# Autodesk Inventor assembly: BV-ASM-222-100
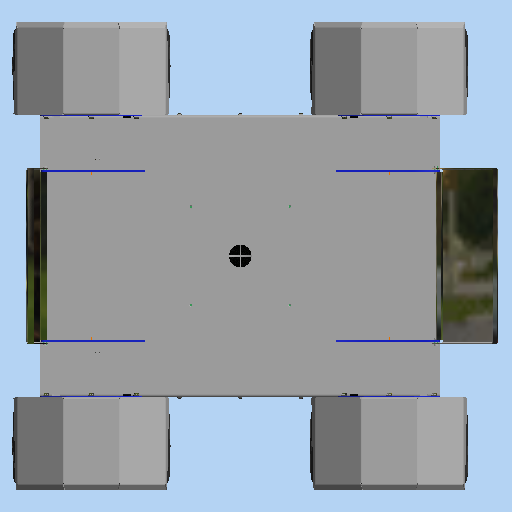
[picture p0: Inventor's stored thumbnail of the model, 512x512]
Saved by Autodesk Inventor 2025.3 (Build 293356030, 356C)
## iProperties
Created: 2025-12-05
Part Number: BV-ASM-222-100
Document SubType Name: Assembly
Designer: josh
Mass: 407870 g
Surface Area: 199043 cm^2
Volume: 211268 cm^3
Density: 1.93058 g/cm^3
Description: BASE VEHICLE COMPLETE ASSEMBLY
Author: josh
## iProperties of the stored document MemberDocs/xFojfi5agHc25u2sk4sonpsnbLc
Created: 2025-12-05
Document SubType Name: Assembly
Designer: josh
Mass: 407870 g
Surface Area: 199043 cm^2
Volume: 211268 cm^3
Density: 1.93058 g/cm^3
Description: BASE VEHICLE COMPLETE ASSEMBLY
Author: josh
## iProperties of the stored document MemberDocs/x54frrunuJ0si20qmEdadrqylTg
Created: 2025-12-05
Document SubType Name: Assembly
Designer: josh
Mass: 407870 g
Surface Area: 199043 cm^2
Volume: 211268 cm^3
Density: 1.93058 g/cm^3
Description: BASE VEHICLE COMPLETE ASSEMBLY
Author: josh
## iProperties of the stored document MemberDocs/xWsksy4mhNck53lhqBkerg4h2Mb
Created: 2025-12-05
Document SubType Name: Assembly
Designer: josh
Mass: 407870 g
Surface Area: 199043 cm^2
Volume: 211268 cm^3
Density: 1.93058 g/cm^3
Description: BASE VEHICLE COMPLETE ASSEMBLY
Author: josh
## Documents named in this file (54)
- R:\A1- Neuweg Design Data\OM Robotics\BASE VEHICLE DESIGN PROJECT\BV-ASM-222-100.iam
- R:\A1- Neuweg Design Data\OM Robotics\BASE VEHICLE DESIGN PROJECT\BV-222-105.ipt
- R:\A1- Neuweg Design Data\OM Robotics\BASE VEHICLE DESIGN PROJECT\BV-222-108.ipt
- R:\A1- Neuweg Design Data\OM Robotics\BASE VEHICLE DESIGN PROJECT\BV-222-112.ipt
- R:\A1- Neuweg Design Data\OM Robotics\BASE VEHICLE DESIGN PROJECT\BV-222-119.ipt
- R:\A1- Neuweg Design Data\OM Robotics\BASE VEHICLE DESIGN PROJECT\BV-222-120.ipt
- R:\A1- Neuweg Design Data\OM Robotics\BASE VEHICLE DESIGN PROJECT\0222-110.ipt
- R:\A1- Neuweg Design Data\OM Robotics\BASE VEHICLE DESIGN PROJECT\3_8-16 x 5_8 Flange Bolt.ipt
- R:\A1- Neuweg Design Data\OM Robotics\BASE VEHICLE DESIGN PROJECT\1_4-20 UNC x 0.625.ipt
- R:\A1- Neuweg Design Data\OM Robotics\BASE VEHICLE DESIGN PROJECT\90128A277.ipt
- R:\A1- Neuweg Design Data\OM Robotics\BASE VEHICLE DESIGN PROJECT\91290A446.ipt
- R:\A1- Neuweg Design Data\OM Robotics\BASE VEHICLE DESIGN PROJECT\91259A177.ipt
- R:\A1- Neuweg Design Data\OM Robotics\BASE VEHICLE DESIGN PROJECT\94945A213.ipt
- R:\A1- Neuweg Design Data\OM Robotics\BASE VEHICLE DESIGN PROJECT\BV-ASM-222-102.iam
- R:\A1- Neuweg Design Data\OM Robotics\BASE VEHICLE DESIGN PROJECT\30205.ipt
- R:\A1- Neuweg Design Data\OM Robotics\BASE VEHICLE DESIGN PROJECT\251105 Motor_Drive.ipt
- R:\A1- Neuweg Design Data\OM Robotics\BASE VEHICLE DESIGN PROJECT\22x10x8.ipt
- R:\A1- Neuweg Design Data\OM Robotics\BASE VEHICLE DESIGN PROJECT\0222-113-2.ipt
- R:\A1- Neuweg Design Data\OM Robotics\BASE VEHICLE DESIGN PROJECT\97260A109.ipt
- R:\A1- Neuweg Design Data\OM Robotics\BASE VEHICLE DESIGN PROJECT\1199N323.ipt
- R:\A1- Neuweg Design Data\OM Robotics\BASE VEHICLE DESIGN PROJECT\BV-ASM-222-103.iam
- R:\A1- Neuweg Design Data\OM Robotics\BASE VEHICLE DESIGN PROJECT\BV-ASM-222-106.iam
- R:\A1- Neuweg Design Data\OM Robotics\BASE VEHICLE DESIGN PROJECT\0222-113.ipt
- R:\A1- Neuweg Design Data\OM Robotics\BASE VEHICLE DESIGN PROJECT\96717A416.ipt
- R:\A1- Neuweg Design Data\OM Robotics\BASE VEHICLE DESIGN PROJECT\4991T961.ipt
- C:\WORK\INVENTOR PROJECTS\misc custom projects\O&M ROBOTICS\ROBOT BASE VEHICLE\BV-222-105.ipt
- C:\WORK\INVENTOR PROJECTS\misc custom projects\O&M ROBOTICS\ROBOT BASE VEHICLE\BV-222-106.ipt
- C:\WORK\INVENTOR PROJECTS\misc custom projects\O&M ROBOTICS\ROBOT BASE VEHICLE\BV-222-107.ipt
- C:\WORK\INVENTOR PROJECTS\misc custom projects\O&M ROBOTICS\ROBOT BASE VEHICLE\BV-222-108.ipt
- C:\WORK\INVENTOR PROJECTS\misc custom projects\O&M ROBOTICS\ROBOT BASE VEHICLE\BV-222-109.ipt
- C:\WORK\INVENTOR PROJECTS\misc custom projects\O&M ROBOTICS\ROBOT BASE VEHICLE\BV-222-112.ipt
- C:\WORK\INVENTOR PROJECTS\misc custom projects\O&M ROBOTICS\ROBOT BASE VEHICLE\BV-222-116.ipt
- C:\WORK\INVENTOR PROJECTS\misc custom projects\O&M ROBOTICS\ROBOT BASE VEHICLE\BV-222-117.ipt
- C:\WORK\INVENTOR PROJECTS\misc custom projects\O&M ROBOTICS\ROBOT BASE VEHICLE\BV-222-118.ipt
- C:\WORK\INVENTOR PROJECTS\misc custom projects\O&M ROBOTICS\ROBOT BASE VEHICLE\BV-222-119.ipt
- C:\WORK\INVENTOR PROJECTS\misc custom projects\O&M ROBOTICS\ROBOT BASE VEHICLE\BV-222-120.ipt
- C:\WORK\INVENTOR PROJECTS\misc custom projects\O&M ROBOTICS\ROBOT BASE VEHICLE\0222-110.ipt
- C:\WORK\INVENTOR PROJECTS\misc custom projects\O&M ROBOTICS\ROBOT BASE VEHICLE\3_8-16 x 5_8 Flange Bolt.ipt
- C:\WORK\INVENTOR PROJECTS\misc custom projects\O&M ROBOTICS\ROBOT BASE VEHICLE\1_4-20 UNC x 0.625.ipt
- C:\WORK\INVENTOR PROJECTS\misc custom projects\O&M ROBOTICS\ROBOT BASE VEHICLE\90128A277\90128A277\90128A277.ipt
- C:\WORK\INVENTOR PROJECTS\misc custom projects\O&M ROBOTICS\ROBOT BASE VEHICLE\91290A446\91290A446\91290A446.ipt
- C:\WORK\INVENTOR PROJECTS\misc custom projects\O&M ROBOTICS\ROBOT BASE VEHICLE\91259A177\91259A177\91259A177.ipt
- C:\WORK\INVENTOR PROJECTS\misc custom projects\O&M ROBOTICS\ROBOT BASE VEHICLE\94945A213\94945A213\94945A213.ipt
- C:\WORK\INVENTOR PROJECTS\misc custom projects\O&M ROBOTICS\ROBOT BASE VEHICLE\BV-ASM-222-102.iam
- C:\WORK\INVENTOR PROJECTS\misc custom projects\O&M ROBOTICS\ROBOT BASE VEHICLE\30205\30205\30205.ipt
- C:\WORK\INVENTOR PROJECTS\misc custom projects\O&M ROBOTICS\ROBOT BASE VEHICLE\251105 Motor_Drive.ipt
- C:\WORK\INVENTOR PROJECTS\misc custom projects\O&M ROBOTICS\ROBOT BASE VEHICLE\22x10x8.ipt
- C:\WORK\INVENTOR PROJECTS\misc custom projects\O&M ROBOTICS\ROBOT BASE VEHICLE\0222-113-2.ipt
- C:\WORK\INVENTOR PROJECTS\misc custom projects\O&M ROBOTICS\ROBOT BASE VEHICLE\97260A109.ipt
- C:\WORK\INVENTOR PROJECTS\misc custom projects\O&M ROBOTICS\ROBOT BASE VEHICLE\93560A112_Steel Hex Weld Nut\93560A112_Steel Hex Weld Nut\93560A112.ipt
- C:\WORK\INVENTOR PROJECTS\misc custom projects\O&M ROBOTICS\ROBOT BASE VEHICLE\1199N323\1199N323\1199N323.ipt
- C:\WORK\INVENTOR PROJECTS\misc custom projects\O&M ROBOTICS\ROBOT BASE VEHICLE\BV-ASM-222-103.iam
- C:\WORK\INVENTOR PROJECTS\misc custom projects\O&M ROBOTICS\ROBOT BASE VEHICLE\BV-ASM-222-104.iam
- C:\WORK\INVENTOR PROJECTS\misc custom projects\O&M ROBOTICS\ROBOT BASE VEHICLE\BV-ASM-222-105.iam
## Components (194 placed, 24 different names)
1. BV-ASM-222-106:1 [sub-assembly] — Insert:95, Insert:96, Insert:97, Insert:98, Insert:99, Insert:100, Insert:101, Insert:102, Insert:103, Insert:104, Insert:129, Insert:130, Insert:131, Insert:132, Insert:133, Insert:134, Insert:135, Insert:136, Insert:137, Insert:138, Insert:139, Insert:140, Insert:141, Insert:142, Insert:143, Insert:144, Mate:105, Mate:107, Mate:108, Mate:109, Mate:111, Mate:113, Mate:114, Mate:116, Mate:118, Mate:120, Mate:122, Mate:123, Mate:124, Insert:221, Insert:222, Insert:223, Mate:125, Mate:126, Mate:127, Insert:226, Insert:227, Insert:228, Mate:128, Mate:129, Mate:130, Insert:231, Insert:232, Insert:233, Mate:131, Mate:132, Mate:133, Insert:234, Insert:235, Insert:236, Flush:20, Mate:134, Insert:238, Insert:240, Mate:136, Insert:243, Insert:244, Insert:245, Insert:246, Insert:247, Insert:248, Insert:249, Insert:250, Insert:252, Insert:253, Insert:254, Insert:255, Insert:256, Insert:257, Insert:258, Insert:259, Insert:260, Insert:261, Insert:262, Insert:263, Insert:264, Insert:265, Insert:266, Insert:267, Insert:268, Insert:269, Insert:270, Insert:271, Insert:272, Insert:273
2. BV-ASM-222-103:1 [sub-assembly] — Flush:8, Flush:9, Flush:10, Mate:131, Mate:132, Mate:133
3. BV-ASM-222-103:2 [sub-assembly] — Insert:205, Insert:206, Mate:128, Mate:129, Mate:130, Insert:229, Insert:230
4. BV-ASM-222-103:3 [sub-assembly] — Insert:209, Insert:210, Mate:125, Mate:126, Mate:127, Insert:224, Insert:225
5. BV-ASM-222-103:4 [sub-assembly] — Insert:213, Insert:214, Mate:122, Mate:123, Mate:124, Insert:219, Insert:220
6. BV-222-105:1 — Insert:117, Insert:118, Insert:119, Insert:120, Insert:121, Insert:122, Insert:123, Insert:124, Insert:125, Insert:126, Insert:127, Insert:128
7. BV-222-108:1 — Flush:1, Mate:3, Mate:135, Mate:136
8. BV-222-112:1 — Mate:73, Mate:74, Mate:75, Mate:76, Mate:77, Mate:78, Mate:79, Mate:80, Mate:81, Mate:82, Mate:83, Mate:84, Mate:85, Mate:86, Mate:87, Mate:88, Mate:89, Mate:90, Mate:91, Mate:92
9. BV-222-119:1 — Insert:175, Insert:190
10. BV-222-120:1 — Mate:5
11. BV-222-112:3
12. BV-222-108:2 — Mate:3, Flush:20, Mate:134, Mate:135
13. BV-222-119:2 — Insert:176, Insert:186
14. BV-222-120:2
15. BV-222-119:3 — Insert:169, Insert:191
16. BV-222-120:3 — Mate:14
17. BV-222-119:4 — Insert:171, Insert:187
18. BV-222-120:4 — Mate:11
19. BV-ASM-222-102:1 [sub-assembly] — Mate:12, Mate:13, Insert:30, Insert:31, Insert:215, Insert:275, Mate:141, Flush:25, Mate:142
20. BV-ASM-222-102:2 [sub-assembly] — Mate:4, Mate:6, Insert:16, Insert:17, Mate:102, Insert:217, Insert:276, Mate:139, Flush:21, Flush:22
21. BV-ASM-222-102:3 [sub-assembly] — Mate:9, Mate:10, Insert:28, Insert:29, Mate:103, Mate:137, Mate:138, Insert:274, Mate:143, Flush:26, Flush:27
22. BV-ASM-222-102:4 [sub-assembly] — Mate:7, Mate:8, Insert:22, Insert:23, Mate:101, Insert:216, Insert:277, Mate:140, Flush:23, Flush:24
23. 251105 Motor_Drive:1 — Mate:4, Mate:5, Mate:6, Flush:2, Flush:3, Mate:102
24. 22x10x8:1 — Insert:16, Insert:17, Insert:280
25. 97260A109:1 — Insert:196
26. 251105 Motor_Drive:2 — Mate:7, Flush:2, Flush:3, Mate:8, Flush:4, Mate:101
27. 97260A109:2 — Insert:194
28. 22x10x8:2 — Insert:22, Insert:23, Insert:281
29. 251105 Motor_Drive:3 — Mate:9, Mate:10, Mate:11, Flush:4, Flush:5, Mate:103
30. 251105 Motor_Drive:4 — Mate:12, Mate:13, Mate:14, Flush:5
31. 97260A109:3 — Insert:200
32. 97260A109:4 — Insert:198
33. 22x10x8:3 — Insert:28, Insert:29, Insert:278
34. 22x10x8:4 — Insert:30, Insert:31, Insert:279
35. 0222-110:1 — Mate:104, Flush:7, Mate:106, Mate:107, Mate:108, Mate:110, Mate:112
36. 0222-110:2 — Flush:7, Flush:19, Mate:113, Mate:115, Mate:117, Mate:119, Mate:121
37. Hex Flange Screw - Inch (IFI) 3/8-16 UNC x 0.625:9 — Mate:120, Mate:121
38. Hex Flange Screw - Inch (IFI) 3/8-16 UNC x 0.625:10 — Mate:118, Mate:119
39. Hex Flange Screw - Inch (IFI) 3/8-16 UNC x 0.625:11 — Mate:116, Mate:117
40. Hex Flange Screw - Inch (IFI) 3/8-16 UNC x 0.625:12 — Mate:114, Mate:115
41. Hex Flange Screw - Inch (IFI) 3/8-16 UNC x 0.625:13 — Mate:105, Mate:106
42. Hex Flange Screw - Inch (IFI) 3/8-16 UNC x 0.625:14 — Mate:109, Mate:110
43. Hex Flange Screw - Inch (IFI) 3/8-16 UNC x 0.625:15
44. Hex Flange Screw - Inch (IFI) 3/8-16 UNC x 0.625:16 — Mate:111, Mate:112
45. Hex Flange Screw - Inch (IFI) 3/8-16 UNC x 0.625:18 — Mate:21, Mate:22, Insert:236
46. Hex Flange Screw - Inch (IFI) 3/8-16 UNC x 0.625:19 — Mate:21, Mate:22, Insert:235
47. Hex Flange Screw - Inch (IFI) 3/8-16 UNC x 0.625:20 — Mate:23, Mate:24, Insert:234
48. Hex Flange Screw - Inch (IFI) 3/8-16 UNC x 0.625:21 — Mate:23, Mate:24, Insert:231
49. Hex Flange Screw - Inch (IFI) 3/8-16 UNC x 0.625:22 — Mate:25, Mate:26, Insert:232
50. Hex Flange Screw - Inch (IFI) 3/8-16 UNC x 0.625:23 — Mate:25, Mate:26, Insert:233
51. Hex Flange Screw - Inch (IFI) 3/8-16 UNC x 0.625:24 — Mate:27, Mate:28, Insert:221
52. Hex Flange Screw - Inch (IFI) 3/8-16 UNC x 0.625:25 — Mate:27, Mate:28, Insert:223
53. Hex Flange Screw - Inch (IFI) 3/8-16 UNC x 0.625:26 — Mate:29, Mate:30, Insert:222
54. Hex Flange Screw - Inch (IFI) 3/8-16 UNC x 0.625:27 — Mate:29, Mate:30, Insert:226
55. Hex Flange Screw - Inch (IFI) 3/8-16 UNC x 0.625:28 — Mate:31, Mate:32, Insert:227
56. Hex Flange Screw - Inch (IFI) 3/8-16 UNC x 0.625:29 — Mate:31, Mate:32, Insert:228
57. Hex Flange Screw - Inch (IFI) 3/8-16 UNC x 0.625:30 — Mate:33, Mate:34
58. Hex Flange Screw - Inch (IFI) 3/8-16 UNC x 0.625:31 — Mate:33, Mate:34
59. Hex Flange Screw - Inch (IFI) 3/8-16 UNC x 0.625:32 — Mate:35, Mate:36, Insert:205, Insert:230
60. Hex Flange Screw - Inch (IFI) 3/8-16 UNC x 0.625:33 — Mate:35, Mate:36, Insert:206, Insert:229
61. Hex Flange Screw - Inch (IFI) 3/8-16 UNC x 0.625:34 — Mate:37, Mate:38, Insert:214, Insert:220
62. Hex Flange Screw - Inch (IFI) 3/8-16 UNC x 0.625:35 — Mate:37, Mate:38, Insert:213, Insert:219
63. Hex Flange Screw - Inch (IFI) 3/8-16 UNC x 0.625:36 — Mate:39, Mate:40, Insert:209, Insert:224
64. Hex Flange Screw - Inch (IFI) 3/8-16 UNC x 0.625:37 — Mate:39, Mate:40, Insert:210, Insert:225
65. 1_4-20 UNC x 0.625:1 — Insert:95, Mate:41, Mate:42
66. 1_4-20 UNC x 0.625:2 — Insert:96, Mate:41, Mate:42
67. 1_4-20 UNC x 0.625:3 — Insert:97, Mate:43, Mate:44
68. 1_4-20 UNC x 0.625:4 — Insert:98, Mate:43, Mate:44
69. 1_4-20 UNC x 0.625:5 — Insert:99, Mate:45, Mate:46
70. 1_4-20 UNC x 0.625:6 — Insert:100, Mate:45, Mate:46
71. 1_4-20 UNC x 0.625:7 — Insert:101, Mate:47, Mate:48
72. 1_4-20 UNC x 0.625:8 — Insert:102, Mate:47, Mate:48
73. 1_4-20 UNC x 0.625:9 — Insert:103, Mate:49, Mate:50
74. 1_4-20 UNC x 0.625:10 — Insert:104, Mate:49, Mate:50
75. Hex Flange Screw - Inch (IFI) 3/8-16 UNC x 0.625:38 — Insert:117, Mate:51, Mate:52
76. Hex Flange Screw - Inch (IFI) 3/8-16 UNC x 0.625:39 — Insert:118, Mate:51, Mate:52
77. Hex Flange Screw - Inch (IFI) 3/8-16 UNC x 0.625:40 — Insert:119, Mate:53, Mate:54
78. Hex Flange Screw - Inch (IFI) 3/8-16 UNC x 0.625:41 — Insert:120, Mate:53, Mate:54
79. Hex Flange Screw - Inch (IFI) 3/8-16 UNC x 0.625:42 — Insert:121, Mate:55, Mate:56
80. Hex Flange Screw - Inch (IFI) 3/8-16 UNC x 0.625:43 — Insert:122, Mate:55, Mate:56
81. Hex Flange Screw - Inch (IFI) 3/8-16 UNC x 0.625:44 — Insert:123, Mate:57, Mate:58
82. Hex Flange Screw - Inch (IFI) 3/8-16 UNC x 0.625:45 — Insert:124, Mate:57, Mate:58
83. Hex Flange Screw - Inch (IFI) 3/8-16 UNC x 0.625:46 — Insert:125, Mate:59, Mate:60
84. Hex Flange Screw - Inch (IFI) 3/8-16 UNC x 0.625:47 — Insert:126, Mate:59, Mate:60
85. Hex Flange Screw - Inch (IFI) 3/8-16 UNC x 0.625:48 — Insert:127, Mate:61, Mate:62
86. Hex Flange Screw - Inch (IFI) 3/8-16 UNC x 0.625:49 — Insert:128, Mate:61, Mate:62
87. 1_4-20 UNC x 0.625:11 — Mate:75, Mate:76
88. 1_4-20 UNC x 0.625:12 — Mate:89, Mate:90
89. 1_4-20 UNC x 0.625:13 — Mate:77, Mate:78
90. 1_4-20 UNC x 0.625:14 — Mate:81, Mate:82
91. 1_4-20 UNC x 0.625:15 — Mate:79, Mate:80
92. 1_4-20 UNC x 0.625:16 — Mate:91, Mate:92
93. 1_4-20 UNC x 0.625:17 — Mate:85, Mate:86
94. 1_4-20 UNC x 0.625:18 — Mate:83, Mate:84
95. 1_4-20 UNC x 0.625:19 — Mate:87, Mate:88
96. 1_4-20 UNC x 0.625:20 — Mate:73, Mate:74
97. 1_4-20 UNC x 0.625:21 — Mate:93, Mate:94
98. 1_4-20 UNC x 0.625:22 — Mate:93, Mate:94
99. 1_4-20 UNC x 0.625:23 — Mate:95, Mate:96
100. 1_4-20 UNC x 0.625:24 — Mate:95, Mate:96
101. 1_4-20 UNC x 0.625:25
102. 1_4-20 UNC x 0.625:26
103. 1_4-20 UNC x 0.625:27 — Mate:97, Mate:98
104. 1_4-20 UNC x 0.625:28 — Mate:97, Mate:98
105. 1_4-20 UNC x 0.625:29 — Mate:99, Mate:100
106. 1_4-20 UNC x 0.625:30 — Mate:99, Mate:100
107. 90128A277:1 — Insert:129
108. 90128A277:2 — Insert:130
109. 90128A277:3 — Insert:131
110. 90128A277:4 — Insert:132
111. 90128A277:5 — Insert:133
112. 90128A277:6 — Insert:134
113. 90128A277:7 — Insert:135
114. 90128A277:8 — Insert:136
115. 90128A277:9 — Insert:137
116. 90128A277:10 — Insert:138
117. 90128A277:11 — Insert:139
118. 90128A277:12 — Insert:140
119. 90128A277:13 — Insert:141
120. 90128A277:14 — Insert:142
121. 90128A277:15 — Insert:143
122. 90128A277:16 — Insert:144
123. 91290A446:1 — Insert:273
124. 91290A446:2 — Insert:271
125. 91290A446:3 — Insert:272
126. 91290A446:4 — Insert:270
127. 91290A446:5 — Insert:260
128. 91290A446:6 — Insert:259
129. 91290A446:7 — Insert:261
130. 91290A446:8 — Insert:258
131. 91290A446:9 — Insert:265
132. 91290A446:10 — Insert:264
133. 91290A446:11 — Insert:262
134. 91290A446:12 — Insert:263
135. 91290A446:13 — Insert:269
136. 91290A446:14 — Insert:268
137. 91290A446:15 — Insert:267
138. 91290A446:16 — Insert:266
139. 91259A177:1 — Insert:244
140. 91259A177:2 — Insert:245
141. 91259A177:3 — Insert:247
142. 91259A177:4 — Insert:248
143. 94945A213:1 — Insert:246
144. 94945A213:2 — Insert:243
145. 94945A213:3 — Insert:238
146. 94945A213:4 — Insert:240
147. 30205:1 — Insert:215, Insert:249
148. 30205:2 — Insert:169, Insert:197
149. 30205:3 — Insert:255, Mate:137, Mate:138
150. 30205:4 — Insert:171, Insert:199
151. 30205:5 — Insert:176, Insert:193
152. 30205:6 — Insert:216, Insert:253
153. 30205:7 — Insert:175, Insert:195
154. 30205:8 — Insert:217, Insert:256
155. 0222-113-2:1 — Insert:199, Insert:200
156. 0222-113-2:2 — Insert:193, Insert:194
157. 0222-113-2:3 — Insert:197, Insert:198
158. 0222-113-2:4 — Insert:195, Insert:196
159. 1199N323:1 — Insert:254
160. 1199N323:2 — Insert:186
161. 1199N323:3 — Insert:187
162. 1199N323:4 — Insert:252
163. 1199N323:5 — Insert:257
164. 1199N323:6 — Insert:190
165. 1199N323:7 — Insert:191
166. 1199N323:8 — Insert:250
167. 0222-113:1 — Insert:274
168. 0222-113:2 — Insert:275
169. 0222-113:3 — Insert:276
170. 0222-113:4 — Insert:277
171. 96717A416:1 — Mate:139, Flush:21, Flush:22
172. 96717A416:2 — Mate:140, Flush:23, Flush:24
173. 96717A416:3 — Mate:141, Flush:25, Mate:142
174. 96717A416:4 — Mate:143, Flush:26, Flush:27
175. 4991T961:1 — Insert:278
176. 4991T961:2
177. 4991T961:3
178. 4991T961:4
179. 4991T961:5
180. 4991T961:6 — Insert:279
181. 4991T961:7
182. 4991T961:8
183. 4991T961:9
184. 4991T961:10
185. 4991T961:11 — Insert:280
186. 4991T961:12
187. 4991T961:13
188. 4991T961:14
189. 4991T961:15
190. 4991T961:16 — Insert:281
191. 4991T961:17
192. 4991T961:18
193. 4991T961:19
194. 4991T961:20
## Component patterns: (5 elements, first: 4991T961:1), (5 elements, first: 4991T961:6), (5 elements, first: 4991T961:11), (5 elements, first: 4991T961:16)
## Relationships (287: Insert 133, Mate 133, Flush 21)
- [Insert]: BV-ASM-222-106:1 ↔ BV-222-112:3
- [Insert]: BV-ASM-222-106:1 ↔ BV-222-112:3
- Flush:1: BV-222-108:1
- Mate:3: BV-222-108:1 ↔ BV-222-108:2
- Mate:4: BV-ASM-222-102:2 ↔ 251105 Motor_Drive:1
- Mate:5: BV-222-120:1 ↔ 251105 Motor_Drive:1
- Mate:6: BV-ASM-222-102:2 ↔ 251105 Motor_Drive:1
- Insert:16: BV-ASM-222-102:2 ↔ 22x10x8:1
- Insert:17: BV-ASM-222-102:2 ↔ 22x10x8:1
- Mate:7: BV-ASM-222-102:4 ↔ 251105 Motor_Drive:2
- Flush:2: 251105 Motor_Drive:1 ↔ 251105 Motor_Drive:2
- Flush:3: 251105 Motor_Drive:1 ↔ 251105 Motor_Drive:2
- Mate:8: BV-ASM-222-102:4 ↔ 251105 Motor_Drive:2
- Insert:22: BV-ASM-222-102:4 ↔ 22x10x8:2
- Insert:23: BV-ASM-222-102:4 ↔ 22x10x8:2
- Mate:9: BV-ASM-222-102:3 ↔ 251105 Motor_Drive:3
- Mate:10: BV-ASM-222-102:3 ↔ 251105 Motor_Drive:3
- Mate:11: BV-222-120:4 ↔ 251105 Motor_Drive:3
- Flush:4: 251105 Motor_Drive:2 ↔ 251105 Motor_Drive:3
- Mate:12: BV-ASM-222-102:1 ↔ 251105 Motor_Drive:4
- Mate:13: BV-ASM-222-102:1 ↔ 251105 Motor_Drive:4
- Mate:14: BV-222-120:3 ↔ 251105 Motor_Drive:4
- Flush:5: 251105 Motor_Drive:3 ↔ 251105 Motor_Drive:4
- Insert:28: BV-ASM-222-102:3 ↔ 22x10x8:3
- Insert:29: BV-ASM-222-102:3 ↔ 22x10x8:3
- Insert:30: BV-ASM-222-102:1 ↔ 22x10x8:4
- Insert:31: BV-ASM-222-102:1 ↔ 22x10x8:4
- Mate:104: 0222-110:1
- Flush:7: 0222-110:1 ↔ 0222-110:2
- Flush:19: 0222-110:2
- Mate:21: Hex Flange Screw - Inch (IFI) 3/8-16 UNC x 0.625:18 ↔ Hex Flange Screw - Inch (IFI) 3/8-16 UNC x 0.625:19
- Mate:22: Hex Flange Screw - Inch (IFI) 3/8-16 UNC x 0.625:18 ↔ Hex Flange Screw - Inch (IFI) 3/8-16 UNC x 0.625:19
- Mate:23: Hex Flange Screw - Inch (IFI) 3/8-16 UNC x 0.625:20 ↔ Hex Flange Screw - Inch (IFI) 3/8-16 UNC x 0.625:21
- Mate:24: Hex Flange Screw - Inch (IFI) 3/8-16 UNC x 0.625:20 ↔ Hex Flange Screw - Inch (IFI) 3/8-16 UNC x 0.625:21
- Mate:25: Hex Flange Screw - Inch (IFI) 3/8-16 UNC x 0.625:22 ↔ Hex Flange Screw - Inch (IFI) 3/8-16 UNC x 0.625:23
- Mate:26: Hex Flange Screw - Inch (IFI) 3/8-16 UNC x 0.625:22 ↔ Hex Flange Screw - Inch (IFI) 3/8-16 UNC x 0.625:23
- Mate:27: Hex Flange Screw - Inch (IFI) 3/8-16 UNC x 0.625:24 ↔ Hex Flange Screw - Inch (IFI) 3/8-16 UNC x 0.625:25
- Mate:28: Hex Flange Screw - Inch (IFI) 3/8-16 UNC x 0.625:24 ↔ Hex Flange Screw - Inch (IFI) 3/8-16 UNC x 0.625:25
- Mate:29: Hex Flange Screw - Inch (IFI) 3/8-16 UNC x 0.625:26 ↔ Hex Flange Screw - Inch (IFI) 3/8-16 UNC x 0.625:27
- Mate:30: Hex Flange Screw - Inch (IFI) 3/8-16 UNC x 0.625:26 ↔ Hex Flange Screw - Inch (IFI) 3/8-16 UNC x 0.625:27
- Mate:31: Hex Flange Screw - Inch (IFI) 3/8-16 UNC x 0.625:28 ↔ Hex Flange Screw - Inch (IFI) 3/8-16 UNC x 0.625:29
- Mate:32: Hex Flange Screw - Inch (IFI) 3/8-16 UNC x 0.625:28 ↔ Hex Flange Screw - Inch (IFI) 3/8-16 UNC x 0.625:29
- [Insert]: BV-ASM-222-103:1 ↔ Hex Flange Screw - Inch (IFI) 3/8-16 UNC x 0.625:30
- [Insert]: BV-ASM-222-103:1 ↔ Hex Flange Screw - Inch (IFI) 3/8-16 UNC x 0.625:31
- Mate:33: Hex Flange Screw - Inch (IFI) 3/8-16 UNC x 0.625:30 ↔ Hex Flange Screw - Inch (IFI) 3/8-16 UNC x 0.625:31
- Mate:34: Hex Flange Screw - Inch (IFI) 3/8-16 UNC x 0.625:30 ↔ Hex Flange Screw - Inch (IFI) 3/8-16 UNC x 0.625:31
- Mate:35: Hex Flange Screw - Inch (IFI) 3/8-16 UNC x 0.625:32 ↔ Hex Flange Screw - Inch (IFI) 3/8-16 UNC x 0.625:33
- Mate:36: Hex Flange Screw - Inch (IFI) 3/8-16 UNC x 0.625:32 ↔ Hex Flange Screw - Inch (IFI) 3/8-16 UNC x 0.625:33
- Mate:37: Hex Flange Screw - Inch (IFI) 3/8-16 UNC x 0.625:34 ↔ Hex Flange Screw - Inch (IFI) 3/8-16 UNC x 0.625:35
- Mate:38: Hex Flange Screw - Inch (IFI) 3/8-16 UNC x 0.625:34 ↔ Hex Flange Screw - Inch (IFI) 3/8-16 UNC x 0.625:35
- Mate:39: Hex Flange Screw - Inch (IFI) 3/8-16 UNC x 0.625:36 ↔ Hex Flange Screw - Inch (IFI) 3/8-16 UNC x 0.625:37
- Mate:40: Hex Flange Screw - Inch (IFI) 3/8-16 UNC x 0.625:36 ↔ Hex Flange Screw - Inch (IFI) 3/8-16 UNC x 0.625:37
- Insert:95: BV-ASM-222-106:1 ↔ 1_4-20 UNC x 0.625:1
- Insert:96: BV-ASM-222-106:1 ↔ 1_4-20 UNC x 0.625:2
- Mate:41: 1_4-20 UNC x 0.625:1 ↔ 1_4-20 UNC x 0.625:2
- Mate:42: 1_4-20 UNC x 0.625:1 ↔ 1_4-20 UNC x 0.625:2
- Insert:97: BV-ASM-222-106:1 ↔ 1_4-20 UNC x 0.625:3
- Insert:98: BV-ASM-222-106:1 ↔ 1_4-20 UNC x 0.625:4
- Mate:43: 1_4-20 UNC x 0.625:3 ↔ 1_4-20 UNC x 0.625:4
- Mate:44: 1_4-20 UNC x 0.625:3 ↔ 1_4-20 UNC x 0.625:4
- Insert:99: BV-ASM-222-106:1 ↔ 1_4-20 UNC x 0.625:5
- Insert:100: BV-ASM-222-106:1 ↔ 1_4-20 UNC x 0.625:6
- Mate:45: 1_4-20 UNC x 0.625:5 ↔ 1_4-20 UNC x 0.625:6
- Mate:46: 1_4-20 UNC x 0.625:5 ↔ 1_4-20 UNC x 0.625:6
- Insert:101: BV-ASM-222-106:1 ↔ 1_4-20 UNC x 0.625:7
- Insert:102: BV-ASM-222-106:1 ↔ 1_4-20 UNC x 0.625:8
- Mate:47: 1_4-20 UNC x 0.625:7 ↔ 1_4-20 UNC x 0.625:8
- Mate:48: 1_4-20 UNC x 0.625:7 ↔ 1_4-20 UNC x 0.625:8
- Insert:103: BV-ASM-222-106:1 ↔ 1_4-20 UNC x 0.625:9
- Insert:104: BV-ASM-222-106:1 ↔ 1_4-20 UNC x 0.625:10
- Mate:49: 1_4-20 UNC x 0.625:9 ↔ 1_4-20 UNC x 0.625:10
- Mate:50: 1_4-20 UNC x 0.625:9 ↔ 1_4-20 UNC x 0.625:10
- Insert:117: BV-222-105:1 ↔ Hex Flange Screw - Inch (IFI) 3/8-16 UNC x 0.625:38
- Insert:118: BV-222-105:1 ↔ Hex Flange Screw - Inch (IFI) 3/8-16 UNC x 0.625:39
- Mate:51: Hex Flange Screw - Inch (IFI) 3/8-16 UNC x 0.625:38 ↔ Hex Flange Screw - Inch (IFI) 3/8-16 UNC x 0.625:39
- Mate:52: Hex Flange Screw - Inch (IFI) 3/8-16 UNC x 0.625:38 ↔ Hex Flange Screw - Inch (IFI) 3/8-16 UNC x 0.625:39
- Insert:119: BV-222-105:1 ↔ Hex Flange Screw - Inch (IFI) 3/8-16 UNC x 0.625:40
- Insert:120: BV-222-105:1 ↔ Hex Flange Screw - Inch (IFI) 3/8-16 UNC x 0.625:41
- Mate:53: Hex Flange Screw - Inch (IFI) 3/8-16 UNC x 0.625:40 ↔ Hex Flange Screw - Inch (IFI) 3/8-16 UNC x 0.625:41
- Mate:54: Hex Flange Screw - Inch (IFI) 3/8-16 UNC x 0.625:40 ↔ Hex Flange Screw - Inch (IFI) 3/8-16 UNC x 0.625:41
- Insert:121: BV-222-105:1 ↔ Hex Flange Screw - Inch (IFI) 3/8-16 UNC x 0.625:42
- Insert:122: BV-222-105:1 ↔ Hex Flange Screw - Inch (IFI) 3/8-16 UNC x 0.625:43
- Mate:55: Hex Flange Screw - Inch (IFI) 3/8-16 UNC x 0.625:42 ↔ Hex Flange Screw - Inch (IFI) 3/8-16 UNC x 0.625:43
- Mate:56: Hex Flange Screw - Inch (IFI) 3/8-16 UNC x 0.625:42 ↔ Hex Flange Screw - Inch (IFI) 3/8-16 UNC x 0.625:43
- Insert:123: BV-222-105:1 ↔ Hex Flange Screw - Inch (IFI) 3/8-16 UNC x 0.625:44
- Insert:124: BV-222-105:1 ↔ Hex Flange Screw - Inch (IFI) 3/8-16 UNC x 0.625:45
- Mate:57: Hex Flange Screw - Inch (IFI) 3/8-16 UNC x 0.625:44 ↔ Hex Flange Screw - Inch (IFI) 3/8-16 UNC x 0.625:45
- Mate:58: Hex Flange Screw - Inch (IFI) 3/8-16 UNC x 0.625:44 ↔ Hex Flange Screw - Inch (IFI) 3/8-16 UNC x 0.625:45
- Insert:125: BV-222-105:1 ↔ Hex Flange Screw - Inch (IFI) 3/8-16 UNC x 0.625:46
- Insert:126: BV-222-105:1 ↔ Hex Flange Screw - Inch (IFI) 3/8-16 UNC x 0.625:47
- Mate:59: Hex Flange Screw - Inch (IFI) 3/8-16 UNC x 0.625:46 ↔ Hex Flange Screw - Inch (IFI) 3/8-16 UNC x 0.625:47
- Mate:60: Hex Flange Screw - Inch (IFI) 3/8-16 UNC x 0.625:46 ↔ Hex Flange Screw - Inch (IFI) 3/8-16 UNC x 0.625:47
- Insert:127: BV-222-105:1 ↔ Hex Flange Screw - Inch (IFI) 3/8-16 UNC x 0.625:48
- Insert:128: BV-222-105:1 ↔ Hex Flange Screw - Inch (IFI) 3/8-16 UNC x 0.625:49
- Mate:61: Hex Flange Screw - Inch (IFI) 3/8-16 UNC x 0.625:48 ↔ Hex Flange Screw - Inch (IFI) 3/8-16 UNC x 0.625:49
- Mate:62: Hex Flange Screw - Inch (IFI) 3/8-16 UNC x 0.625:48 ↔ Hex Flange Screw - Inch (IFI) 3/8-16 UNC x 0.625:49
- [Mate]: 1_4-20 UNC x 0.625:11 ↔ 1_4-20 UNC x 0.625:12
- [Mate]: 1_4-20 UNC x 0.625:11 ↔ 1_4-20 UNC x 0.625:12
- [Mate]: 1_4-20 UNC x 0.625:13 ↔ 1_4-20 UNC x 0.625:14
- [Mate]: 1_4-20 UNC x 0.625:13 ↔ 1_4-20 UNC x 0.625:14
- [Mate]: 1_4-20 UNC x 0.625:17 ↔ 1_4-20 UNC x 0.625:18
- [Mate]: 1_4-20 UNC x 0.625:17 ↔ 1_4-20 UNC x 0.625:18
- [Mate]: 1_4-20 UNC x 0.625:19 ↔ 1_4-20 UNC x 0.625:20
- [Mate]: 1_4-20 UNC x 0.625:19 ↔ 1_4-20 UNC x 0.625:20
- Mate:73: BV-222-112:1 ↔ 1_4-20 UNC x 0.625:20
- Mate:74: BV-222-112:1 ↔ 1_4-20 UNC x 0.625:20
- Mate:75: BV-222-112:1 ↔ 1_4-20 UNC x 0.625:11
- Mate:76: BV-222-112:1 ↔ 1_4-20 UNC x 0.625:11
- Mate:77: BV-222-112:1 ↔ 1_4-20 UNC x 0.625:13
- Mate:78: BV-222-112:1 ↔ 1_4-20 UNC x 0.625:13
- Mate:79: BV-222-112:1 ↔ 1_4-20 UNC x 0.625:15
- Mate:80: BV-222-112:1 ↔ 1_4-20 UNC x 0.625:15
- Mate:81: BV-222-112:1 ↔ 1_4-20 UNC x 0.625:14
- Mate:82: BV-222-112:1 ↔ 1_4-20 UNC x 0.625:14
- Mate:83: BV-222-112:1 ↔ 1_4-20 UNC x 0.625:18
- Mate:84: BV-222-112:1 ↔ 1_4-20 UNC x 0.625:18
- Mate:85: BV-222-112:1 ↔ 1_4-20 UNC x 0.625:17
- Mate:86: BV-222-112:1 ↔ 1_4-20 UNC x 0.625:17
- Mate:87: BV-222-112:1 ↔ 1_4-20 UNC x 0.625:19
- Mate:88: BV-222-112:1 ↔ 1_4-20 UNC x 0.625:19
- Mate:89: BV-222-112:1 ↔ 1_4-20 UNC x 0.625:12
- Mate:90: BV-222-112:1 ↔ 1_4-20 UNC x 0.625:12
- Mate:91: BV-222-112:1 ↔ 1_4-20 UNC x 0.625:16
- Mate:92: BV-222-112:1 ↔ 1_4-20 UNC x 0.625:16
- Mate:93: 1_4-20 UNC x 0.625:21 ↔ 1_4-20 UNC x 0.625:22
- Mate:94: 1_4-20 UNC x 0.625:21 ↔ 1_4-20 UNC x 0.625:22
- Mate:95: 1_4-20 UNC x 0.625:23 ↔ 1_4-20 UNC x 0.625:24
- Mate:96: 1_4-20 UNC x 0.625:23 ↔ 1_4-20 UNC x 0.625:24
- Mate:97: 1_4-20 UNC x 0.625:27 ↔ 1_4-20 UNC x 0.625:28
- Mate:98: 1_4-20 UNC x 0.625:27 ↔ 1_4-20 UNC x 0.625:28
- Mate:99: 1_4-20 UNC x 0.625:29 ↔ 1_4-20 UNC x 0.625:30
- Mate:100: 1_4-20 UNC x 0.625:29 ↔ 1_4-20 UNC x 0.625:30
- Insert:129: BV-ASM-222-106:1 ↔ 90128A277:1
- Insert:130: BV-ASM-222-106:1 ↔ 90128A277:2
- Insert:131: BV-ASM-222-106:1 ↔ 90128A277:3
- Insert:132: BV-ASM-222-106:1 ↔ 90128A277:4
- Insert:133: BV-ASM-222-106:1 ↔ 90128A277:5
- Insert:134: BV-ASM-222-106:1 ↔ 90128A277:6
- Insert:135: BV-ASM-222-106:1 ↔ 90128A277:7
- Insert:136: BV-ASM-222-106:1 ↔ 90128A277:8
- Insert:137: BV-ASM-222-106:1 ↔ 90128A277:9
- Insert:138: BV-ASM-222-106:1 ↔ 90128A277:10
- Insert:139: BV-ASM-222-106:1 ↔ 90128A277:11
- Insert:140: BV-ASM-222-106:1 ↔ 90128A277:12
- Insert:141: BV-ASM-222-106:1 ↔ 90128A277:13
- Insert:142: BV-ASM-222-106:1 ↔ 90128A277:14
- Insert:143: BV-ASM-222-106:1 ↔ 90128A277:15
- Insert:144: BV-ASM-222-106:1 ↔ 90128A277:16
- Insert:169: BV-222-119:3 ↔ 30205:2
- Insert:171: BV-222-119:4 ↔ 30205:4
- Insert:175: BV-222-119:1 ↔ 30205:7
- Insert:176: BV-222-119:2 ↔ 30205:5
- Insert:186: BV-222-119:2 ↔ 1199N323:2
- Insert:187: BV-222-119:4 ↔ 1199N323:3
- Insert:190: BV-222-119:1 ↔ 1199N323:6
- Insert:191: BV-222-119:3 ↔ 1199N323:7
- Insert:193: 30205:5 ↔ 0222-113-2:2
- Insert:194: 97260A109:2 ↔ 0222-113-2:2
- Insert:195: 30205:7 ↔ 0222-113-2:4
- Insert:196: 97260A109:1 ↔ 0222-113-2:4
- Insert:197: 30205:2 ↔ 0222-113-2:3
- Insert:198: 97260A109:4 ↔ 0222-113-2:3
- Insert:199: 30205:4 ↔ 0222-113-2:1
- Insert:200: 97260A109:3 ↔ 0222-113-2:1
- Flush:8: BV-ASM-222-103:1
- Flush:9: BV-ASM-222-103:1
- Flush:10: BV-ASM-222-103:1
- Insert:205: BV-ASM-222-103:2 ↔ Hex Flange Screw - Inch (IFI) 3/8-16 UNC x 0.625:32
- Insert:206: BV-ASM-222-103:2 ↔ Hex Flange Screw - Inch (IFI) 3/8-16 UNC x 0.625:33
- Insert:209: BV-ASM-222-103:3 ↔ Hex Flange Screw - Inch (IFI) 3/8-16 UNC x 0.625:36
- Insert:210: BV-ASM-222-103:3 ↔ Hex Flange Screw - Inch (IFI) 3/8-16 UNC x 0.625:37
- Insert:213: BV-ASM-222-103:4 ↔ Hex Flange Screw - Inch (IFI) 3/8-16 UNC x 0.625:35
- Insert:214: BV-ASM-222-103:4 ↔ Hex Flange Screw - Inch (IFI) 3/8-16 UNC x 0.625:34
- [Flush]: BV-ASM-222-106:1
- [Flush]: BV-ASM-222-106:1
- [Flush]: BV-ASM-222-106:1
- Insert:215: BV-ASM-222-102:1 ↔ 30205:1
- Mate:101: BV-ASM-222-102:4 ↔ 251105 Motor_Drive:2
- Insert:216: BV-ASM-222-102:4 ↔ 30205:6
- Mate:102: BV-ASM-222-102:2 ↔ 251105 Motor_Drive:1
- Insert:217: BV-ASM-222-102:2 ↔ 30205:8
- Mate:103: BV-ASM-222-102:3 ↔ 251105 Motor_Drive:3
- Mate:105: BV-ASM-222-106:1 ↔ Hex Flange Screw - Inch (IFI) 3/8-16 UNC x 0.625:13
- Mate:106: 0222-110:1 ↔ Hex Flange Screw - Inch (IFI) 3/8-16 UNC x 0.625:13
- Mate:107: BV-ASM-222-106:1 ↔ 0222-110:1
- Mate:108: BV-ASM-222-106:1 ↔ 0222-110:1
- Mate:109: BV-ASM-222-106:1 ↔ Hex Flange Screw - Inch (IFI) 3/8-16 UNC x 0.625:14
- Mate:110: 0222-110:1 ↔ Hex Flange Screw - Inch (IFI) 3/8-16 UNC x 0.625:14
- Mate:111: BV-ASM-222-106:1 ↔ Hex Flange Screw - Inch (IFI) 3/8-16 UNC x 0.625:16
- Mate:112: 0222-110:1 ↔ Hex Flange Screw - Inch (IFI) 3/8-16 UNC x 0.625:16
- Mate:113: BV-ASM-222-106:1 ↔ 0222-110:2
- Mate:114: BV-ASM-222-106:1 ↔ Hex Flange Screw - Inch (IFI) 3/8-16 UNC x 0.625:12
- Mate:115: 0222-110:2 ↔ Hex Flange Screw - Inch (IFI) 3/8-16 UNC x 0.625:12
- Mate:116: BV-ASM-222-106:1 ↔ Hex Flange Screw - Inch (IFI) 3/8-16 UNC x 0.625:11
- Mate:117: 0222-110:2 ↔ Hex Flange Screw - Inch (IFI) 3/8-16 UNC x 0.625:11
- Mate:118: BV-ASM-222-106:1 ↔ Hex Flange Screw - Inch (IFI) 3/8-16 UNC x 0.625:10
- Mate:119: 0222-110:2 ↔ Hex Flange Screw - Inch (IFI) 3/8-16 UNC x 0.625:10
- Mate:120: BV-ASM-222-106:1 ↔ Hex Flange Screw - Inch (IFI) 3/8-16 UNC x 0.625:9
- Mate:121: 0222-110:2 ↔ Hex Flange Screw - Inch (IFI) 3/8-16 UNC x 0.625:9
- Mate:122: BV-ASM-222-106:1 ↔ BV-ASM-222-103:4
- Mate:123: BV-ASM-222-106:1 ↔ BV-ASM-222-103:4
- Mate:124: BV-ASM-222-106:1 ↔ BV-ASM-222-103:4
- Insert:219: BV-ASM-222-103:4 ↔ Hex Flange Screw - Inch (IFI) 3/8-16 UNC x 0.625:35
- Insert:220: BV-ASM-222-103:4 ↔ Hex Flange Screw - Inch (IFI) 3/8-16 UNC x 0.625:34
- Insert:221: BV-ASM-222-106:1 ↔ Hex Flange Screw - Inch (IFI) 3/8-16 UNC x 0.625:24
- Insert:222: BV-ASM-222-106:1 ↔ Hex Flange Screw - Inch (IFI) 3/8-16 UNC x 0.625:26
- Insert:223: BV-ASM-222-106:1 ↔ Hex Flange Screw - Inch (IFI) 3/8-16 UNC x 0.625:25
- Mate:125: BV-ASM-222-106:1 ↔ BV-ASM-222-103:3
- Mate:126: BV-ASM-222-106:1 ↔ BV-ASM-222-103:3
- Mate:127: BV-ASM-222-106:1 ↔ BV-ASM-222-103:3
- Insert:224: BV-ASM-222-103:3 ↔ Hex Flange Screw - Inch (IFI) 3/8-16 UNC x 0.625:36
- Insert:225: BV-ASM-222-103:3 ↔ Hex Flange Screw - Inch (IFI) 3/8-16 UNC x 0.625:37
- Insert:226: BV-ASM-222-106:1 ↔ Hex Flange Screw - Inch (IFI) 3/8-16 UNC x 0.625:27
- Insert:227: BV-ASM-222-106:1 ↔ Hex Flange Screw - Inch (IFI) 3/8-16 UNC x 0.625:28
- Insert:228: BV-ASM-222-106:1 ↔ Hex Flange Screw - Inch (IFI) 3/8-16 UNC x 0.625:29
- Mate:128: BV-ASM-222-106:1 ↔ BV-ASM-222-103:2
- Mate:129: BV-ASM-222-106:1 ↔ BV-ASM-222-103:2
- Mate:130: BV-ASM-222-106:1 ↔ BV-ASM-222-103:2
- Insert:229: BV-ASM-222-103:2 ↔ Hex Flange Screw - Inch (IFI) 3/8-16 UNC x 0.625:33
- Insert:230: BV-ASM-222-103:2 ↔ Hex Flange Screw - Inch (IFI) 3/8-16 UNC x 0.625:32
- Insert:231: BV-ASM-222-106:1 ↔ Hex Flange Screw - Inch (IFI) 3/8-16 UNC x 0.625:21
- Insert:232: BV-ASM-222-106:1 ↔ Hex Flange Screw - Inch (IFI) 3/8-16 UNC x 0.625:22
- Insert:233: BV-ASM-222-106:1 ↔ Hex Flange Screw - Inch (IFI) 3/8-16 UNC x 0.625:23
- Mate:131: BV-ASM-222-106:1 ↔ BV-ASM-222-103:1
- Mate:132: BV-ASM-222-106:1 ↔ BV-ASM-222-103:1
- Mate:133: BV-ASM-222-106:1 ↔ BV-ASM-222-103:1
- Insert:234: BV-ASM-222-106:1 ↔ Hex Flange Screw - Inch (IFI) 3/8-16 UNC x 0.625:20
- Insert:235: BV-ASM-222-106:1 ↔ Hex Flange Screw - Inch (IFI) 3/8-16 UNC x 0.625:19
- Insert:236: BV-ASM-222-106:1 ↔ Hex Flange Screw - Inch (IFI) 3/8-16 UNC x 0.625:18
- Flush:20: BV-ASM-222-106:1 ↔ BV-222-108:2
- Mate:134: BV-ASM-222-106:1 ↔ BV-222-108:2
- Insert:238: BV-ASM-222-106:1 ↔ 94945A213:3
- Insert:240: BV-ASM-222-106:1 ↔ 94945A213:4
- Mate:135: BV-222-108:1 ↔ BV-222-108:2
- Mate:136: BV-ASM-222-106:1 ↔ BV-222-108:1
- Insert:243: BV-ASM-222-106:1 ↔ 94945A213:2
- Insert:244: BV-ASM-222-106:1 ↔ 91259A177:1
- Insert:245: BV-ASM-222-106:1 ↔ 91259A177:2
- Insert:246: BV-ASM-222-106:1 ↔ 94945A213:1
- Insert:247: BV-ASM-222-106:1 ↔ 91259A177:3
- Insert:248: BV-ASM-222-106:1 ↔ 91259A177:4
- Insert:249: BV-ASM-222-106:1 ↔ 30205:1
- Insert:250: BV-ASM-222-106:1 ↔ 1199N323:8
- Insert:252: BV-ASM-222-106:1 ↔ 1199N323:4
- Insert:253: BV-ASM-222-106:1 ↔ 30205:6
- Insert:254: BV-ASM-222-106:1 ↔ 1199N323:1
- Insert:255: BV-ASM-222-106:1 ↔ 30205:3
- Insert:256: BV-ASM-222-106:1 ↔ 30205:8
- Insert:257: BV-ASM-222-106:1 ↔ 1199N323:5
- Insert:258: BV-ASM-222-106:1 ↔ 91290A446:8
- Insert:259: BV-ASM-222-106:1 ↔ 91290A446:6
- Insert:260: BV-ASM-222-106:1 ↔ 91290A446:5
- Insert:261: BV-ASM-222-106:1 ↔ 91290A446:7
- Insert:262: BV-ASM-222-106:1 ↔ 91290A446:11
- Insert:263: BV-ASM-222-106:1 ↔ 91290A446:12
- Insert:264: BV-ASM-222-106:1 ↔ 91290A446:10
- Insert:265: BV-ASM-222-106:1 ↔ 91290A446:9
- Insert:266: BV-ASM-222-106:1 ↔ 91290A446:16
- Insert:267: BV-ASM-222-106:1 ↔ 91290A446:15
- Insert:268: BV-ASM-222-106:1 ↔ 91290A446:14
- Insert:269: BV-ASM-222-106:1 ↔ 91290A446:13
- Insert:270: BV-ASM-222-106:1 ↔ 91290A446:4
- Insert:271: BV-ASM-222-106:1 ↔ 91290A446:2
- Insert:272: BV-ASM-222-106:1 ↔ 91290A446:3
- Insert:273: BV-ASM-222-106:1 ↔ 91290A446:1
- Mate:137: BV-ASM-222-102:3 ↔ 30205:3
- Mate:138: BV-ASM-222-102:3 ↔ 30205:3
- Insert:274: BV-ASM-222-102:3 ↔ 0222-113:1
- Insert:275: BV-ASM-222-102:1 ↔ 0222-113:2
- Insert:276: BV-ASM-222-102:2 ↔ 0222-113:3
- Insert:277: BV-ASM-222-102:4 ↔ 0222-113:4
- Mate:139: BV-ASM-222-102:2 ↔ 96717A416:1
- Flush:21: BV-ASM-222-102:2 ↔ 96717A416:1
- Flush:22: BV-ASM-222-102:2 ↔ 96717A416:1
- Mate:140: BV-ASM-222-102:4 ↔ 96717A416:2
- Flush:23: BV-ASM-222-102:4 ↔ 96717A416:2
- Flush:24: BV-ASM-222-102:4 ↔ 96717A416:2
- Mate:141: BV-ASM-222-102:1 ↔ 96717A416:3
- Flush:25: BV-ASM-222-102:1 ↔ 96717A416:3
- Mate:142: BV-ASM-222-102:1 ↔ 96717A416:3
- Mate:143: BV-ASM-222-102:3 ↔ 96717A416:4
- Flush:26: BV-ASM-222-102:3 ↔ 96717A416:4
- Flush:27: BV-ASM-222-102:3 ↔ 96717A416:4
- Insert:278: 22x10x8:3 ↔ 4991T961:1
- Insert:279: 22x10x8:4 ↔ 4991T961:6
- Insert:280: 22x10x8:1 ↔ 4991T961:11
- Insert:281: 22x10x8:2 ↔ 4991T961:16
## Named parameters: d214_d160 = 0 mm, d215_d161 = 0 mm, d216_d164 = 0 mm, d217_d165 = 0 mm, d220_d172 = 0 mm, d221_d173 = 0 mm, d222_d176 = 0 mm, d223_d177 = 0 mm
